# Autodesk Inventor assembly: wheel-assembly
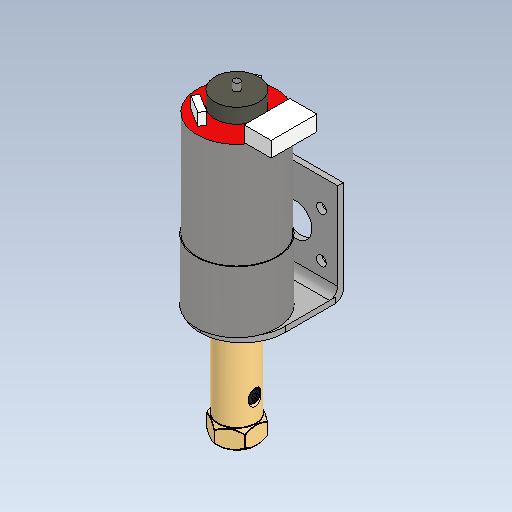
[picture p0: Inventor's stored thumbnail of the model, 512x512]
Saved by Autodesk Inventor 2025 (Build 290162000, 162)
## iProperties
Created: 2025-08-20
Part Number: wheel-assembly
Document SubType Name: Assembly
Designer: HP
Author: HP
## Documents named in this file (4)
- C:\Users\HP\Documents\GitHub\robotics-dojo-2025\CAD\wheel-assembly.iam
- C:\Users\HP\Documents\GitHub\robotics-dojo-2025\CAD\motor\JGA25-370 DC12V350RPM.ipt
- C:\Users\HP\Documents\GitHub\robotics-dojo-2025\CAD\bracket\MOTA_SuporteJGA v3.ipt
- C:\Users\HP\Documents\GitHub\robotics-dojo-2025\CAD\coupling\Hexagonal Brass Shaft Coupling Motor Transmission Connector v2.iam
## Components (3 placed, 3 different names)
1. JGA25-370 DC12V350RPM:1 — Mate:1, Insert:1, Mate:5, Mate:6, Mate:7, Angle:1
2. MOTA_SuporteJGA v3:1 — Mate:1, Insert:1, Angle:1
3. Hexagonal Brass Shaft Coupling Motor Transmission Connector v2:1 [sub-assembly] — Mate:5, Mate:6, Mate:7
## Relationships (6: Mate 4, Insert 1, Angle 1)
- Mate:1: JGA25-370 DC12V350RPM:1 ↔ MOTA_SuporteJGA v3:1
- Insert:1: JGA25-370 DC12V350RPM:1 ↔ MOTA_SuporteJGA v3:1
- Mate:5: JGA25-370 DC12V350RPM:1 ↔ Hexagonal Brass Shaft Coupling Motor Transmission Connector v2:1
- Mate:6: JGA25-370 DC12V350RPM:1 ↔ Hexagonal Brass Shaft Coupling Motor Transmission Connector v2:1
- Mate:7 (2 mm): JGA25-370 DC12V350RPM:1 ↔ Hexagonal Brass Shaft Coupling Motor Transmission Connector v2:1
- Angle:1 (90 deg): JGA25-370 DC12V350RPM:1 ↔ MOTA_SuporteJGA v3:1
